# Autodesk Inventor assembly: Ensamblaje carcasa control
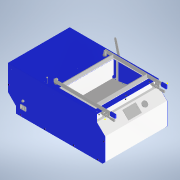
[picture p0: Inventor's stored thumbnail of the model, 180x180]
Saved by Autodesk Inventor 2021 (Build 250183000, 183)
## iProperties
Created: 2021-04-15
Part Number: Ensamblaje carcasa control
Document SubType Name: Assembly
Designer: Admin
Author: Admin
## Documents named in this file (22)
- D:\Nelson\Documentos\Inventor\PAI_ElementosInternos\Ensamblaje carcasa control.iam
- D:\Nelson\Documentos\Inventor\PAI_ElementosInternos\Carcasa_azul.ipt
- D:\Nelson\Documentos\Inventor\PAI_ElementosInternos\Carcaza_blanca_frontal.ipt
- D:\Nelson\Documentos\Inventor\PAI_ElementosInternos\Tapa_blanca_inferior.ipt
- D:\Nelson\Documentos\Inventor\PAI_ElementosInternos\Vacuometro.ipt
- D:\Nelson\Documentos\Inventor\PAI_ElementosInternos\HMI_NV3W_MR20L_V1.iam
- D:\Nelson\Documentos\Inventor\PAI_ElementosInternos\Receptaculo e interruptor.ipt
- D:\Nelson\Documentos\Inventor\PAI_ElementosInternos\Portafusible para fusible de 13A.ipt
- D:\Nelson\Documentos\Inventor\PAI_ElementosInternos\Tapa_interior_1.ipt
- D:\Nelson\Documentos\Inventor\PAI_ElementosInternos\Tapa_interior_2.ipt
- D:\Nelson\Documentos\Inventor\PAI_ElementosInternos\Tapa_blanca_trasera.ipt
- D:\Nelson\Documentos\Inventor\PAI_ElementosInternos\Bomba de Vacio.ipt
- D:\Nelson\Documentos\Inventor\PAI_ElementosInternos\Marco molde.ipt
- D:\Nelson\Documentos\Inventor\PAI_ElementosInternos\CSN 02 1721 - 17,5.ipt
- D:\Nelson\Documentos\Inventor\PAI_ElementosInternos\Ensamblaje_soportme molde_barras.iam
- D:\Nelson\Documentos\Inventor\PAI_ElementosInternos\Mecanismo Modelado.iam
- D:\Nelson\Documentos\Inventor\PAI_ElementosInternos\Bandeja_proteccion_carcasa_control.ipt
- D:\Nelson\Documentos\Inventor\PAI_ElementosInternos\BS 4320 - M5 (Forma A).ipt
- D:\Nelson\Documentos\Inventor\PAI_ElementosInternos\ISO 7380-1 - M5 x 8.ipt
- D:\Nelson\Documentos\Inventor\PAI_ElementosInternos\BS 4183 - M5(1).ipt
- D:\Nelson\Documentos\Inventor\PAI_ElementosInternos\MecanismoBoqueoCarro\ProtectorBloqueo.ipt
- D:\Nelson\Documentos\Inventor\PAI_ElementosInternos\Ensamble eléctrico.iam
## Components (76 placed, 21 different names)
1. Carcasa_azul:1 — Coincidencia:1, Nivelación:1, Coincidencia:2, Coincidencia:3, Nivelación:2, Coincidencia:5, Coincidencia:6, Coincidencia:7, Coincidencia:8, Coincidencia:9, Coincidencia:18, Coincidencia:20, Coincidencia:27, Nivelación:6, Nivelación:7, Coincidencia:28, Coincidencia:29, Coincidencia:30, Coincidencia:31, Coincidencia:32, Coincidencia:34, Nivelación:8, Nivelación:9, Coincidencia:35, De rotación:1, De rotación:2, De rotación:4, De rotación:5, De rotación:6, De rotación:7, De rotación:8, De rotación:9, De rotación:10, De rotación:11, De rotación:42, De rotación:48, De rotación:64, De rotación:65, De rotación:66, Coincidencia:36, Mate:38, Coincidencia:39, Rígido:2
2. Carcaza_blanca_frontal:1 — Coincidencia:1, Nivelación:1, Coincidencia:2, Coincidencia:4, Coincidencia:10, Coincidencia:11, Coincidencia:12, Coincidencia:13, Coincidencia:14, Coincidencia:19, De rotación:24, De rotación:25, De rotación:26, De rotación:56, De rotación:57, De rotación:58, De rotación:70, De rotación:71, De rotación:72
3. Tapa_blanca_inferior:1 — Coincidencia:3, Coincidencia:4, Nivelación:2, Nivelación:4, Coincidencia:21, Mate:25, Flush:5, Mate:26, De rotación:38, De rotación:39, De rotación:40, De rotación:41, De rotación:44, De rotación:45, De rotación:46, De rotación:49, De rotación:50, De rotación:51, De rotación:52, Mate:40
4. Vacuometro:1 — Coincidencia:10, Coincidencia:11
5. HMI_NV3W_MR20L_V1:1 [sub-assembly] — Coincidencia:12, Coincidencia:13, Coincidencia:14
6. Receptaculo e interruptor:1 — Coincidencia:7, Coincidencia:8, Coincidencia:9
7. Portafusible para fusible de 13A:1 — Coincidencia:5, Coincidencia:6
8. Tapa_interior_2:1 — Coincidencia:18, Coincidencia:19, De rotación:62, De rotación:63, Rígido:1
9. Tapa_blanca_trasera:1 — Coincidencia:20, Nivelación:4, Coincidencia:21
10. Bomba de Vacio:1 — Mate:25, Flush:5, Mate:26
11. Marco molde:1 — Coincidencia:27, Nivelación:6, Nivelación:7
12. CSN 02 1721 17,5:1 — Coincidencia:28, Coincidencia:30, Cilíndrica:1
13. CSN 02 1721 17,5:2 — Coincidencia:29, Coincidencia:31
14. Ensamblaje_soportme molde_barras:1 [sub-assembly] — Cilíndrica:1
15. Mecanismo Modelado:1 [sub-assembly] — Coincidencia:32, Coincidencia:34, Coincidencia:36, Mate:37
16. Bandeja_proteccion_carcasa_control:1 — Nivelación:8, Nivelación:9, Coincidencia:35
17. BS 4320 Forma AB M5 (Forma A):4 — De rotación:1, De rotación:16
18. BS 4320 Forma AB M5 (Forma A):5 — De rotación:2, De rotación:15
19. BS 4320 Forma AB M5 (Forma A):7 — De rotación:4, De rotación:14
20. BS 4320 Forma AB M5 (Forma A):8 — De rotación:5, De rotación:17
21. BS 4320 Forma AB M5 (Forma A):9 — De rotación:6, De rotación:13
22. BS 4320 Forma AB M5 (Forma A):10 — De rotación:9, De rotación:21
23. BS 4320 Forma AB M5 (Forma A):11 — De rotación:7, De rotación:23
24. BS 4320 Forma AB M5 (Forma A):12 — De rotación:11, De rotación:19
25. BS 4320 Forma AB M5 (Forma A):13 — De rotación:8, De rotación:22
26. BS 4320 Forma AB M5 (Forma A):14 — De rotación:10, De rotación:20
27. ISO 7380-1 M5 x 8:1 — De rotación:15
28. ISO 7380-1 M5 x 8:3 — De rotación:17
29. ISO 7380-1 M5 x 8:4 — De rotación:16
30. ISO 7380-1 M5 x 8:5 — De rotación:14
31. ISO 7380-1 M5 x 8:6 — De rotación:13
32. ISO 7380-1 M5 x 8:7 — De rotación:20
33. ISO 7380-1 M5 x 8:8 — De rotación:21
34. ISO 7380-1 M5 x 8:10 — De rotación:23
35. ISO 7380-1 M5 x 8:11 — De rotación:19
36. ISO 7380-1 M5 x 8:12 — De rotación:22
37. ISO 7380-1 M5 x 8:13 — De rotación:27
38. ISO 7380-1 M5 x 8:14 — De rotación:29
39. ISO 7380-1 M5 x 8:15 — De rotación:28
40. BS 4320 Forma AB M5 (Forma A):16 — De rotación:26, De rotación:27
41. BS 4320 Forma AB M5 (Forma A):17 — De rotación:25, De rotación:28
42. BS 4320 Forma AB M5 (Forma A):18 — De rotación:24, De rotación:29
43. BS 4183 - Métrico M5:1 — De rotación:38
44. BS 4183 - Métrico M5:2 — De rotación:39
45. BS 4183 - Métrico M5:3 — De rotación:42
46. BS 4183 - Métrico M5:4 — De rotación:40
47. BS 4183 - Métrico M5:6 — De rotación:41
48. BS 4183 - Métrico M5:7 — De rotación:45
49. BS 4183 - Métrico M5:8 — De rotación:44
50. BS 4183 - Métrico M5:10 — De rotación:46
51. BS 4183 - Métrico M5:11 — De rotación:48
52. BS 4183 - Métrico M5:12 — De rotación:49
53. BS 4183 - Métrico M5:13 — De rotación:50
54. BS 4183 - Métrico M5:14 — De rotación:52
55. BS 4183 - Métrico M5:15 — De rotación:51
56. ISO 7380-1 M5 x 8:21 — De rotación:59
57. ISO 7380-1 M5 x 8:22 — De rotación:60
58. ISO 7380-1 M5 x 8:23 — De rotación:61
59. BS 4320 Forma AB M5 (Forma A):22 — De rotación:57, De rotación:60
60. BS 4320 Forma AB M5 (Forma A):23 — De rotación:58, De rotación:61
61. BS 4320 Forma AB M5 (Forma A):24 — De rotación:56, De rotación:59
62. BS 4183 - Métrico M5:19 — De rotación:62
63. BS 4183 - Métrico M5:20 — De rotación:63
64. BS 4183 - Métrico M5:21 — Rígido:1
65. ISO 7380-1 M5 x 8:24 — De rotación:69
66. ISO 7380-1 M5 x 8:25 — De rotación:68
67. ISO 7380-1 M5 x 8:26 — De rotación:67
68. BS 4320 Forma AB M5 (Forma A):25 — De rotación:66, De rotación:69
69. BS 4320 Forma AB M5 (Forma A):26 — De rotación:65, De rotación:68
70. BS 4320 Forma AB M5 (Forma A):27 — De rotación:64, De rotación:67
71. BS 4183 - Métrico M5:22 — De rotación:70
72. BS 4183 - Métrico M5:23 — De rotación:72
73. BS 4183 - Métrico M5:24 — De rotación:71
74. ProtectorBloqueo:1 — Mate:37, Mate:38
75. Tapa_interior_1:1 — Coincidencia:39, Rígido:2
76. Ensamble eléctrico:1 [sub-assembly] — Mate:40
## Relationships (100: RevoluteJoint 56, Mate 33, Flush 8, WeldJoint 2, CylindricalJoint 1)
- Coincidencia:1 [Mate]: Carcasa_azul:1 ↔ Carcaza_blanca_frontal:1
- Nivelación:1 [Flush]: Carcasa_azul:1 ↔ Carcaza_blanca_frontal:1
- Coincidencia:2 [Mate]: Carcasa_azul:1 ↔ Carcaza_blanca_frontal:1
- Coincidencia:3 [Mate]: Carcasa_azul:1 ↔ Tapa_blanca_inferior:1
- Coincidencia:4 [Mate]: Carcaza_blanca_frontal:1 ↔ Tapa_blanca_inferior:1
- Nivelación:2 [Flush]: Carcasa_azul:1 ↔ Tapa_blanca_inferior:1
- Coincidencia:5 [Mate]: Carcasa_azul:1 ↔ Portafusible para fusible de 13A:1
- Coincidencia:6 [Mate]: Carcasa_azul:1 ↔ Portafusible para fusible de 13A:1
- Coincidencia:7 [Mate]: Carcasa_azul:1 ↔ Receptaculo e interruptor:1
- Coincidencia:8 [Mate]: Carcasa_azul:1 ↔ Receptaculo e interruptor:1
- Coincidencia:9 [Mate]: Carcasa_azul:1 ↔ Receptaculo e interruptor:1
- Coincidencia:10 [Mate]: Carcaza_blanca_frontal:1 ↔ Vacuometro:1
- Coincidencia:11 [Mate]: Carcaza_blanca_frontal:1 ↔ Vacuometro:1
- Coincidencia:12 [Mate]: Carcaza_blanca_frontal:1 ↔ HMI_NV3W_MR20L_V1:1
- Coincidencia:13 [Mate]: Carcaza_blanca_frontal:1 ↔ HMI_NV3W_MR20L_V1:1
- Coincidencia:14 [Mate]: Carcaza_blanca_frontal:1 ↔ HMI_NV3W_MR20L_V1:1
- Coincidencia:18 [Mate]: Carcasa_azul:1 ↔ Tapa_interior_2:1
- Coincidencia:19 [Mate]: Carcaza_blanca_frontal:1 ↔ Tapa_interior_2:1
- Coincidencia:20 [Mate]: Carcasa_azul:1 ↔ Tapa_blanca_trasera:1
- Nivelación:4 [Flush]: Tapa_blanca_inferior:1 ↔ Tapa_blanca_trasera:1
- Coincidencia:21 [Mate]: Tapa_blanca_inferior:1 ↔ Tapa_blanca_trasera:1
- Mate:25: Tapa_blanca_inferior:1 ↔ Bomba de Vacio:1
- Flush:5 (30 mm): Tapa_blanca_inferior:1 ↔ Bomba de Vacio:1
- Mate:26 (130 mm): Tapa_blanca_inferior:1 ↔ Bomba de Vacio:1
- Coincidencia:27 [Mate]: Carcasa_azul:1 ↔ Marco molde:1
- Nivelación:6 [Flush]: Carcasa_azul:1 ↔ Marco molde:1
- Nivelación:7 [Flush]: Carcasa_azul:1 ↔ Marco molde:1
- Coincidencia:28 [Mate]: Carcasa_azul:1 ↔ CSN 02 1721 17,5:1
- Coincidencia:29 [Mate]: Carcasa_azul:1 ↔ CSN 02 1721 17,5:2
- Coincidencia:30 [Mate]: Carcasa_azul:1 ↔ CSN 02 1721 17,5:1
- Coincidencia:31 [Mate]: Carcasa_azul:1 ↔ CSN 02 1721 17,5:2
- Cilíndrica:1 [CylindricalJoint]: CSN 02 1721 17,5:1 ↔ Ensamblaje_soportme molde_barras:1
- Coincidencia:32 [Mate]: Carcasa_azul:1 ↔ Mecanismo Modelado:1
- Coincidencia:34 [Mate]: Carcasa_azul:1 ↔ Mecanismo Modelado:1
- Nivelación:8 [Flush] (5 mm): Carcasa_azul:1 ↔ Bandeja_proteccion_carcasa_control:1
- Nivelación:9 [Flush]: Carcasa_azul:1 ↔ Bandeja_proteccion_carcasa_control:1
- Coincidencia:35 [Mate]: Carcasa_azul:1 ↔ Bandeja_proteccion_carcasa_control:1
- De rotación:1 [RevoluteJoint]: Carcasa_azul:1 ↔ BS 4320 Forma AB M5 (Forma A):4
- De rotación:2 [RevoluteJoint]: Carcasa_azul:1 ↔ BS 4320 Forma AB M5 (Forma A):5
- De rotación:4 [RevoluteJoint]: Carcasa_azul:1 ↔ BS 4320 Forma AB M5 (Forma A):7
- De rotación:5 [RevoluteJoint]: Carcasa_azul:1 ↔ BS 4320 Forma AB M5 (Forma A):8
- De rotación:6 [RevoluteJoint]: Carcasa_azul:1 ↔ BS 4320 Forma AB M5 (Forma A):9
- De rotación:7 [RevoluteJoint]: Carcasa_azul:1 ↔ BS 4320 Forma AB M5 (Forma A):11
- De rotación:8 [RevoluteJoint]: Carcasa_azul:1 ↔ BS 4320 Forma AB M5 (Forma A):13
- De rotación:9 [RevoluteJoint]: Carcasa_azul:1 ↔ BS 4320 Forma AB M5 (Forma A):10
- De rotación:10 [RevoluteJoint]: Carcasa_azul:1 ↔ BS 4320 Forma AB M5 (Forma A):14
- De rotación:11 [RevoluteJoint]: Carcasa_azul:1 ↔ BS 4320 Forma AB M5 (Forma A):12
- De rotación:13 [RevoluteJoint]: BS 4320 Forma AB M5 (Forma A):9 ↔ ISO 7380-1 M5 x 8:6
- De rotación:14 [RevoluteJoint]: BS 4320 Forma AB M5 (Forma A):7 ↔ ISO 7380-1 M5 x 8:5
- De rotación:15 [RevoluteJoint]: BS 4320 Forma AB M5 (Forma A):5 ↔ ISO 7380-1 M5 x 8:1
- De rotación:16 [RevoluteJoint]: BS 4320 Forma AB M5 (Forma A):4 ↔ ISO 7380-1 M5 x 8:4
- De rotación:17 [RevoluteJoint]: BS 4320 Forma AB M5 (Forma A):8 ↔ ISO 7380-1 M5 x 8:3
- De rotación:19 [RevoluteJoint]: BS 4320 Forma AB M5 (Forma A):12 ↔ ISO 7380-1 M5 x 8:11
- De rotación:20 [RevoluteJoint]: BS 4320 Forma AB M5 (Forma A):14 ↔ ISO 7380-1 M5 x 8:7
- De rotación:21 [RevoluteJoint]: BS 4320 Forma AB M5 (Forma A):10 ↔ ISO 7380-1 M5 x 8:8
- De rotación:22 [RevoluteJoint]: BS 4320 Forma AB M5 (Forma A):13 ↔ ISO 7380-1 M5 x 8:12
- De rotación:23 [RevoluteJoint]: BS 4320 Forma AB M5 (Forma A):11 ↔ ISO 7380-1 M5 x 8:10
- De rotación:24 [RevoluteJoint]: Carcaza_blanca_frontal:1 ↔ BS 4320 Forma AB M5 (Forma A):18
- De rotación:25 [RevoluteJoint]: Carcaza_blanca_frontal:1 ↔ BS 4320 Forma AB M5 (Forma A):17
- De rotación:26 [RevoluteJoint]: Carcaza_blanca_frontal:1 ↔ BS 4320 Forma AB M5 (Forma A):16
- De rotación:27 [RevoluteJoint]: ISO 7380-1 M5 x 8:13 ↔ BS 4320 Forma AB M5 (Forma A):16
- De rotación:28 [RevoluteJoint]: ISO 7380-1 M5 x 8:15 ↔ BS 4320 Forma AB M5 (Forma A):17
- De rotación:29 [RevoluteJoint]: ISO 7380-1 M5 x 8:14 ↔ BS 4320 Forma AB M5 (Forma A):18
- De rotación:38 [RevoluteJoint]: Tapa_blanca_inferior:1 ↔ BS 4183 - Métrico M5:1
- De rotación:39 [RevoluteJoint]: Tapa_blanca_inferior:1 ↔ BS 4183 - Métrico M5:2
- De rotación:40 [RevoluteJoint]: Tapa_blanca_inferior:1 ↔ BS 4183 - Métrico M5:4
- De rotación:41 [RevoluteJoint]: Tapa_blanca_inferior:1 ↔ BS 4183 - Métrico M5:6
- De rotación:42 [RevoluteJoint]: Carcasa_azul:1 ↔ BS 4183 - Métrico M5:3
- De rotación:44 [RevoluteJoint]: Tapa_blanca_inferior:1 ↔ BS 4183 - Métrico M5:8
- De rotación:45 [RevoluteJoint]: Tapa_blanca_inferior:1 ↔ BS 4183 - Métrico M5:7
- De rotación:46 [RevoluteJoint]: Tapa_blanca_inferior:1 ↔ BS 4183 - Métrico M5:10
- De rotación:48 [RevoluteJoint]: Carcasa_azul:1 ↔ BS 4183 - Métrico M5:11
- De rotación:49 [RevoluteJoint]: Tapa_blanca_inferior:1 ↔ BS 4183 - Métrico M5:12
- De rotación:50 [RevoluteJoint]: Tapa_blanca_inferior:1 ↔ BS 4183 - Métrico M5:13
- De rotación:51 [RevoluteJoint]: Tapa_blanca_inferior:1 ↔ BS 4183 - Métrico M5:15
- De rotación:52 [RevoluteJoint]: Tapa_blanca_inferior:1 ↔ BS 4183 - Métrico M5:14
- De rotación:56 [RevoluteJoint]: Carcaza_blanca_frontal:1 ↔ BS 4320 Forma AB M5 (Forma A):24
- De rotación:57 [RevoluteJoint]: Carcaza_blanca_frontal:1 ↔ BS 4320 Forma AB M5 (Forma A):22
- De rotación:58 [RevoluteJoint]: Carcaza_blanca_frontal:1 ↔ BS 4320 Forma AB M5 (Forma A):23
- De rotación:59 [RevoluteJoint]: ISO 7380-1 M5 x 8:21 ↔ BS 4320 Forma AB M5 (Forma A):24
- De rotación:60 [RevoluteJoint]: ISO 7380-1 M5 x 8:22 ↔ BS 4320 Forma AB M5 (Forma A):22
- De rotación:61 [RevoluteJoint]: ISO 7380-1 M5 x 8:23 ↔ BS 4320 Forma AB M5 (Forma A):23
- De rotación:62 [RevoluteJoint]: Tapa_interior_2:1 ↔ BS 4183 - Métrico M5:19
- De rotación:63 [RevoluteJoint]: Tapa_interior_2:1 ↔ BS 4183 - Métrico M5:20
- Rígido:1 [WeldJoint]: Tapa_interior_2:1 ↔ BS 4183 - Métrico M5:21
- De rotación:64 [RevoluteJoint]: Carcasa_azul:1 ↔ BS 4320 Forma AB M5 (Forma A):27
- De rotación:65 [RevoluteJoint]: Carcasa_azul:1 ↔ BS 4320 Forma AB M5 (Forma A):26
- De rotación:66 [RevoluteJoint]: Carcasa_azul:1 ↔ BS 4320 Forma AB M5 (Forma A):25
- De rotación:67 [RevoluteJoint]: ISO 7380-1 M5 x 8:26 ↔ BS 4320 Forma AB M5 (Forma A):27
- De rotación:68 [RevoluteJoint]: ISO 7380-1 M5 x 8:25 ↔ BS 4320 Forma AB M5 (Forma A):26
- De rotación:69 [RevoluteJoint]: ISO 7380-1 M5 x 8:24 ↔ BS 4320 Forma AB M5 (Forma A):25
- De rotación:70 [RevoluteJoint]: Carcaza_blanca_frontal:1 ↔ BS 4183 - Métrico M5:22
- De rotación:71 [RevoluteJoint]: Carcaza_blanca_frontal:1 ↔ BS 4183 - Métrico M5:24
- De rotación:72 [RevoluteJoint]: Carcaza_blanca_frontal:1 ↔ BS 4183 - Métrico M5:23
- Coincidencia:36 [Mate]: Carcasa_azul:1 ↔ Mecanismo Modelado:1
- Mate:37: Mecanismo Modelado:1 ↔ ProtectorBloqueo:1
- Mate:38: Carcasa_azul:1 ↔ ProtectorBloqueo:1
- Coincidencia:39 [Mate]: Carcasa_azul:1 ↔ Tapa_interior_1:1
- Rígido:2 [WeldJoint]: Carcasa_azul:1 ↔ Tapa_interior_1:1
- Mate:40: Tapa_blanca_inferior:1 ↔ Ensamble eléctrico:1
